# Autodesk Inventor assembly: MotorBlockTwoWheels
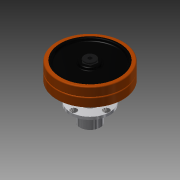
[picture p0: Inventor's stored thumbnail of the model, 180x180]
Saved by Autodesk Inventor 2014 SP1 (Build 180222100, 222)
## iProperties
Created: 2015-04-11
Part Number: MotorBlockTwoWheels
Document SubType Name: Assembly
Designer: david
Author: david
## Documents named in this file (3)
- C:\Users\asus\Documents\Autodesk\Projects\AUSBEEDone\Components\Motors\MotorBlockTwoWheels.iam
- C:\Users\asus\Documents\Autodesk\Projects\AUSBEEDone\Components\BaneBots\TwoWheelsBlock.iam
- C:\Users\asus\Documents\Autodesk\Projects\AUSBEEDone\Components\Motors\Motor.iam
## Components (2 placed, 2 different names)
1. TwoWheelsBlock:1 [sub-assembly] — Mate:1, Mate:2, Angle:1
2. Motor:1 [sub-assembly] — Mate:1, Mate:2, Angle:1
## Relationships (3: Mate 2, Angle 1)
- Mate:1: TwoWheelsBlock:1 ↔ Motor:1
- Mate:2: TwoWheelsBlock:1 ↔ Motor:1
- Angle:1 (0 deg): TwoWheelsBlock:1 ↔ Motor:1
